# Autodesk Inventor assembly: NS-01-17_IGUS-Führung
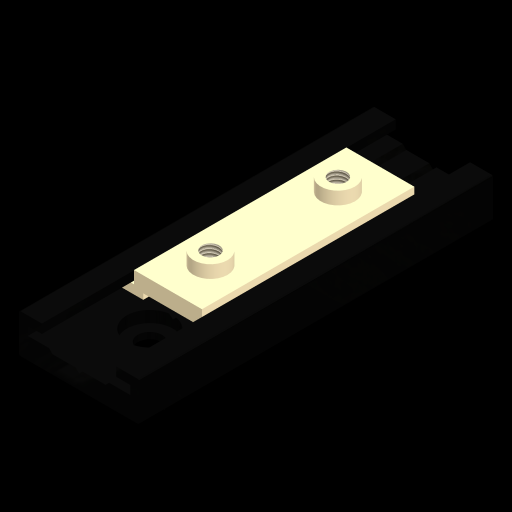
[picture p0: Inventor's stored thumbnail of the model, 512x512]
Saved by Autodesk Inventor 2024 (Build 280153000, 153)
## iProperties
Created: 2023-10-20
Part Number: NS-01-17_IGUS-Führung
Document SubType Name: Assembly
Designer: buchmannmartin
Author: buchmannmartin
## Documents named in this file (3)
- E:\User\Dokumente\#BeneEspressoscope\NS-01-17_IGUS-Führung.iam
- E:\User\Dokumente\#BeneEspressoscope\IGUS-NS-01-17x50.ipt
- E:\User\Dokumente\#BeneEspressoscope\IGUS-NW-22-17-30.ipt
## Components (2 placed, 2 different names)
1. IGUS-NS-01-17x50:1 — Passend:1, Fluchtend:1
2. IGUS-NW-22-17-30:1 — Passend:1, Fluchtend:1
## Relationships (2: Mate 1, Flush 1)
- Passend:1 [Mate]: IGUS-NS-01-17x50:1 ↔ IGUS-NW-22-17-30:1
- Fluchtend:1 [Flush]: IGUS-NS-01-17x50:1 ↔ IGUS-NW-22-17-30:1
